# Autodesk Inventor assembly: KB33-046-000 -РобоПатруль.txt
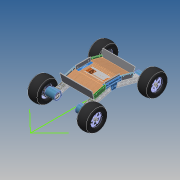
[picture p0: Inventor's stored thumbnail of the model, 180x180]
Saved by Autodesk Inventor 2020 (Build 240168000, 168)
## iProperties
Created: 2021-06-08
Part Number: KB33-046-000 -РобоПатруль.txt
Material: Типовые
Document SubType Name: Assembly
Designer: Петров Иван
Mass: 5533.39 g
Surface Area: 11164.5 cm^2
Volume: 5565.55 cm^3
Density: 0.994223 g/cm^3
Author: Петров Иван
## Documents named in this file (3)
- E:\IVAN\Ivan_desktop\Kvantorium\Projects\RoboPatrol\design\KB33-046-000 - РобоПатруль.iam
- E:\IVAN\Ivan_desktop\Kvantorium\Projects\RoboPatrol\design\KB33-046-001 - Ходовая часть.iam
- E:\IVAN\Ivan_desktop\Kvantorium\Projects\RoboPatrol\design\KB33-046-004 - Внешний корпус.iam
## Components (2 placed, 2 different names)
1. KB33-046-001 - Ходовая часть:1 [sub-assembly] — Совмещение:1, Совмещение:2, Совмещение:3
2. KB33-046-004 - Внешний корпус:1 [sub-assembly] — Совмещение:1, Совмещение:2, Совмещение:3
## Relationships (3: Mate 3)
- Совмещение:1 [Mate]: KB33-046-001 - Ходовая часть:1 ↔ KB33-046-004 - Внешний корпус:1
- Совмещение:2 [Mate]: KB33-046-001 - Ходовая часть:1 ↔ KB33-046-004 - Внешний корпус:1
- Совмещение:3 [Mate]: KB33-046-001 - Ходовая часть:1 ↔ KB33-046-004 - Внешний корпус:1
